# Autodesk Inventor assembly: suportes_anti_empenamento
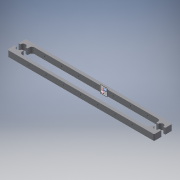
[picture p0: Inventor's stored thumbnail of the model, 180x180]
Saved by Autodesk Inventor 2018 (Build 220112000, 112)
## iProperties
Created: 2018-08-15
Part Number: suportes_anti_empenamento
Material: Genérico
Document SubType Name: Assembly
Designer: Georgines
Author: Georgines
## Documents named in this file (2)
- C:\Users\Georgines\Documents\EstacaoBGA\Peças 3D\Usinagem\suportes_anti_empenamento.iam
- C:\Users\Georgines\Documents\EstacaoBGA\Peças 3D\SuporteAntiEmpenamento.ipt
## Components (2 placed, 1 different names)
1. SuporteAntiEmpenamento:1 — Coincidência:1, Alinhamento:1, Alinhamento:2
2. SuporteAntiEmpenamento:2 — Coincidência:1, Alinhamento:1, Alinhamento:2
## Relationships (3: Flush 2, Mate 1)
- Coincidência:1 [Mate] (29 mm): SuporteAntiEmpenamento:1 ↔ SuporteAntiEmpenamento:2
- Alinhamento:1 [Flush]: SuporteAntiEmpenamento:1 ↔ SuporteAntiEmpenamento:2
- Alinhamento:2 [Flush]: SuporteAntiEmpenamento:1 ↔ SuporteAntiEmpenamento:2
